# Autodesk Inventor assembly: main_assembly
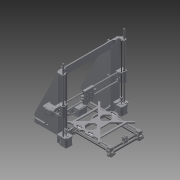
[picture p0: Inventor's stored thumbnail of the model, 180x180]
Saved by Autodesk Inventor 2015 SP2 (Build 190223200, 223)
## iProperties
Created: 2015-05-09
Part Number: main_assembly
Document SubType Name: Assembly
Designer: X
Author: X
## Documents named in this file (22)
- C:\Users\marc\Documents\GitHub\Prusa_i3\main_assembly.iam
- C:\Users\marc\Documents\GitHub\Prusa_i3\frame\platform_redrawn.ipt
- C:\Users\marc\Documents\GitHub\Prusa_i3\3d_printer_part\y-belt-holder.ipt
- C:\Users\marc\Documents\GitHub\Prusa_i3\chassis.iam
- C:\Users\marc\Documents\GitHub\Prusa_i3\Imported Components\NEMA 17 Stepper Motor Assembly\NEMA 17 Stepper Motor Assembly.iam
- C:\Users\marc\Documents\GitHub\Prusa_i3\standard_parts\LM8UU 8mm Linear Bearing.ipt
- C:\Users\marc\Documents\GitHub\Prusa_i3\main_frame_assem.iam
- C:\Users\marc\Documents\GitHub\Prusa_i3\standard_parts\ISO 7093 A\ISO 7093 A - ST 10 - 140 HV .ipt
- C:\Users\marc\Documents\GitHub\Prusa_i3\standard_parts\DIN 934\DIN 934 - M10 x 1.5.ipt
- C:\Users\marc\Documents\GitHub\Prusa_i3\standard_parts\DIN 84\DIN 84 - M3 x 16.ipt
- C:\Users\marc\Documents\GitHub\Prusa_i3\standard_parts\DIN 7985 (H)\DIN 7985 (H) - M3x18-H.ipt
- C:\Users\marc\Documents\GitHub\Prusa_i3\standard_parts\DIN 7985 (H)\DIN 7985 (H) - M3x16-H.ipt
- C:\Users\marc\Documents\GitHub\Prusa_i3\standard_parts\DIN 934\DIN 934 - M3.5 x 0.6.ipt
- C:\Users\marc\Documents\GitHub\Prusa_i3\Imported Components\coupler\coupler.ipt
- C:\Users\marc\Documents\GitHub\Prusa_i3\rod\smooth_rod_z_axis.ipt
- C:\Users\marc\Documents\GitHub\Prusa_i3\rod\threaded_rod_z_axis.ipt
- C:\Users\marc\Documents\GitHub\Prusa_i3\3d_printer_part\x-end-motor.ipt
- C:\Users\marc\Documents\GitHub\Prusa_i3\3d_printer_part\x-end-idler.ipt
- C:\Users\marc\Documents\GitHub\Prusa_i3\rod\smooth_rod_x_axis.ipt
- C:\Users\marc\Documents\GitHub\Prusa_i3\3d_printer_part\x-carriage.ipt
- C:\Users\marc\Documents\GitHub\Prusa_i3\frame\support1.ipt
- C:\Users\marc\Documents\GitHub\Prusa_i3\frame\support2.ipt
## Components (66 placed, 21 different names)
1. platform_redrawn:1 — Cylindrical:1, Cylindrical:2, Mate:1, Angle:1, Mate:3, Tangent:1, Tangent:2, Mate:4, Mate:5, Mate:27
2. y-belt-holder:1 — Cylindrical:1, Cylindrical:2, Mate:1
3. chassis:1 [sub-assembly] — Cylindrical:3, Cylindrical:4, Mate:2, Cylindrical:5, Cylindrical:6, Cylindrical:7, Angle:1, Mate:6, Mate:7, Cylindrical:8, Cylindrical:9, Cylindrical:10, Cylindrical:11, Cylindrical:12, Cylindrical:13, Cylindrical:14, Cylindrical:15, Cylindrical:16, Cylindrical:17, Mate:27, Flush:1, Mate:30
4. NEMA 17 Stepper Motor Assembly:1 [sub-assembly] — Cylindrical:3, Cylindrical:4, Mate:2
5. LM8UU 8mm Linear Bearing:1 — Cylindrical:6, Mate:3, Tangent:1, Tangent:2
6. LM8UU 8mm Linear Bearing:2 — Cylindrical:5, Mate:4
7. LM8UU 8mm Linear Bearing:3 — Cylindrical:7, Mate:5
8. main_frame_assem:1 [sub-assembly] — Cylindrical:8, Cylindrical:9, Mate:8, Mate:9, Mate:10, Mate:11, Mate:16, Cylindrical:18, Mate:17, Cylindrical:19, Mate:18, Cylindrical:20, Insert:1, Insert:2, Insert:3, Mate:19, Cylindrical:21, Mate:20, Cylindrical:22, Cylindrical:23, Mate:21, Mate:22, Mate:23, Mate:24, Mate:25, Mate:26, Insert:4, Insert:5, Insert:6, Insert:7, Insert:8, Insert:9, Insert:10, Insert:11, Insert:12, Insert:13, Insert:14, Insert:15, Insert:16, Insert:17, Insert:18, Insert:19, Insert:20, Cylindrical:26, Cylindrical:27, Mate:30, Mate:38, Mate:39, Mate:40, Mate:41, Mate:42, Mate:43
9. ISO 7093 A ST 10 - 140 HV - A:1 — Cylindrical:12, Mate:9, Mate:12
10. ISO 7093 A ST 10 - 140 HV - A:2 — Cylindrical:13, Mate:10, Mate:13
11. ISO 7093 A ST 10 - 140 HV - A:3 — Cylindrical:10, Mate:8, Mate:15
12. ISO 7093 A ST 10 - 140 HV - A:4 — Cylindrical:11, Mate:11, Mate:14
13. DIN 934 - replaced by DIN EN 24032/28673/28674 M10:1 — Cylindrical:14, Mate:12
14. DIN 934 - replaced by DIN EN 24032/28673/28674 M10:2 — Cylindrical:15, Mate:13
15. DIN 934 - replaced by DIN EN 24032/28673/28674 M10:3 — Cylindrical:17, Mate:15
16. DIN 934 - replaced by DIN EN 24032/28673/28674 M10:4 — Cylindrical:16, Mate:14
17. DIN 84 - replaced by DIN EN ISO 1207 M3 x 16:1 — Mate:16, Cylindrical:18
18. DIN 84 - replaced by DIN EN ISO 1207 M3 x 16:2 — Mate:17, Cylindrical:19
19. DIN 84 - replaced by DIN EN ISO 1207 M3 x 16:3 — Mate:18, Cylindrical:20
20. DIN 84 - replaced by DIN EN ISO 1207 M3 x 16:4 — Insert:1
21. DIN 84 - replaced by DIN EN ISO 1207 M3 x 16:5 — Insert:2
22. DIN 84 - replaced by DIN EN ISO 1207 M3 x 16:6 — Insert:3
23. NEMA 17 Stepper Motor Assembly:2 [sub-assembly] — Mate:19, Cylindrical:21, Cylindrical:24, Cylindrical:25, Mate:28, Mate:31, Mate:34
24. NEMA 17 Stepper Motor Assembly:3 [sub-assembly] — Mate:20, Cylindrical:22, Cylindrical:23, Mate:29, Cylindrical:28, Mate:32, Mate:33
25. DIN 7985 (H) M3x18-H:1 — Mate:21, Mate:22
26. DIN 7985 (H) M3x18-H:2 — Mate:23, Mate:24
27. DIN 7985 (H) M3x18-H:3 — Mate:25, Mate:26, Cylindrical:25
28. DIN 7985 (H) M3x18-H:4 — Insert:4
29. DIN 7985 (H) M3x18-H:5 — Insert:5
30. DIN 7985 (H) M3x18-H:6 — Insert:6
31. DIN 7985 (H) M3x16-H:1 — Insert:7
32. DIN 7985 (H) M3x16-H:2 — Insert:8
33. DIN 7985 (H) M3x16-H:3 — Insert:9
34. DIN 7985 (H) M3x16-H:4 — Insert:10
35. DIN 934 - replaced by DIN EN 24032/28673/28674 M3.5:1 — Insert:11
36. DIN 934 - replaced by DIN EN 24032/28673/28674 M3.5:2 — Insert:12
37. DIN 934 - replaced by DIN EN 24032/28673/28674 M3.5:3 — Insert:13
38. DIN 934 - replaced by DIN EN 24032/28673/28674 M3.5:4 — Insert:14
39. DIN 934 - replaced by DIN EN 24032/28673/28674 M3.5:5 — Insert:15
40. DIN 934 - replaced by DIN EN 24032/28673/28674 M3.5:6 — Insert:16
41. DIN 934 - replaced by DIN EN 24032/28673/28674 M3.5:7 — Insert:17
42. DIN 934 - replaced by DIN EN 24032/28673/28674 M3.5:8 — Insert:18
43. DIN 934 - replaced by DIN EN 24032/28673/28674 M3.5:9 — Insert:19
44. DIN 934 - replaced by DIN EN 24032/28673/28674 M3.5:10 — Insert:20
45. coupler:1 — Cylindrical:24, Mate:31, Cylindrical:30
46. smooth_rod_z_axis:1 — Cylindrical:26, Mate:28, Cylindrical:39
47. smooth_rod_z_axis:2 — Cylindrical:27, Mate:29, Cylindrical:35
48. coupler:2 — Cylindrical:28, Mate:32, Cylindrical:29
49. threaded_rod_z_axis:1 — Mate:33, Cylindrical:29, Cylindrical:37
50. threaded_rod_z_axis:2 — Mate:34, Cylindrical:30, Cylindrical:40
51. x-end-idler:1 — Cylindrical:33, Cylindrical:34, Flush:4, Flush:5, Cylindrical:35, Cylindrical:37, Cylindrical:41, Cylindrical:42, Mate:35, Mate:36
52. LM8UU 8mm Linear Bearing:4 — Cylindrical:32, Cylindrical:38, Flush:6, Cylindrical:39
53. LM8UU 8mm Linear Bearing:5 — Cylindrical:32, Flush:7
54. LM8UU 8mm Linear Bearing:6 — Cylindrical:34, Flush:4
55. LM8UU 8mm Linear Bearing:7 — Cylindrical:33, Flush:5
56. x-end-motor:1 — Cylindrical:38, Flush:6, Flush:7, Cylindrical:40, Cylindrical:43, Cylindrical:44, Mate:37, Cylindrical:45, Cylindrical:46
57. smooth_rod_x_axis:1 — Cylindrical:41, Cylindrical:44, Mate:35, Cylindrical:51
58. smooth_rod_x_axis:2 — Cylindrical:42, Cylindrical:43, Mate:36, Cylindrical:52
59. NEMA 17 Stepper Motor Assembly:4 [sub-assembly] — Mate:37, Cylindrical:45, Cylindrical:46
60. x-carriage:1 — Cylindrical:47, Cylindrical:48, Cylindrical:49, Cylindrical:50, Flush:8, Flush:9, Flush:10, Flush:11, Cylindrical:51, Cylindrical:52
61. LM8UU 8mm Linear Bearing:8 — Cylindrical:47, Flush:9
62. LM8UU 8mm Linear Bearing:9 — Cylindrical:48, Flush:8
63. LM8UU 8mm Linear Bearing:10 — Cylindrical:49, Flush:10
64. LM8UU 8mm Linear Bearing:11 — Cylindrical:50, Flush:11
65. support1:1 — Mate:38, Mate:39, Mate:40
66. support2:1 — Mate:41, Mate:42, Mate:43
## Relationships (125: CylindricalJoint 50, Mate 43, Insert 20, Flush 9, Tangent 2, Angle 1)
- Cylindrical:1: platform_redrawn:1 ↔ y-belt-holder:1
- Cylindrical:2: platform_redrawn:1 ↔ y-belt-holder:1
- Mate:1: platform_redrawn:1 ↔ y-belt-holder:1
- Cylindrical:3: chassis:1 ↔ NEMA 17 Stepper Motor Assembly:1
- Cylindrical:4: chassis:1 ↔ NEMA 17 Stepper Motor Assembly:1
- Mate:2: chassis:1 ↔ NEMA 17 Stepper Motor Assembly:1
- Cylindrical:5: chassis:1 ↔ LM8UU 8mm Linear Bearing:2
- Cylindrical:6: chassis:1 ↔ LM8UU 8mm Linear Bearing:1
- Cylindrical:7: chassis:1 ↔ LM8UU 8mm Linear Bearing:3
- Angle:1 (0 deg): platform_redrawn:1 ↔ chassis:1
- Mate:3 (3.5 mm): platform_redrawn:1 ↔ LM8UU 8mm Linear Bearing:1
- Tangent:1: platform_redrawn:1 ↔ LM8UU 8mm Linear Bearing:1
- Tangent:2: platform_redrawn:1 ↔ LM8UU 8mm Linear Bearing:1
- Mate:4 (3.5 mm): platform_redrawn:1 ↔ LM8UU 8mm Linear Bearing:2
- Mate:5 (3.5 mm): platform_redrawn:1 ↔ LM8UU 8mm Linear Bearing:3
- Mate:6: chassis:1
- Mate:7: chassis:1
- Cylindrical:8: chassis:1 ↔ main_frame_assem:1
- Cylindrical:9: chassis:1 ↔ main_frame_assem:1
- Cylindrical:10: chassis:1 ↔ ISO 7093 A ST 10 - 140 HV - A:3
- Cylindrical:11: chassis:1 ↔ ISO 7093 A ST 10 - 140 HV - A:4
- Cylindrical:12: chassis:1 ↔ ISO 7093 A ST 10 - 140 HV - A:1
- Cylindrical:13: chassis:1 ↔ ISO 7093 A ST 10 - 140 HV - A:2
- Mate:8: main_frame_assem:1 ↔ ISO 7093 A ST 10 - 140 HV - A:3
- Mate:9: main_frame_assem:1 ↔ ISO 7093 A ST 10 - 140 HV - A:1
- Mate:10: main_frame_assem:1 ↔ ISO 7093 A ST 10 - 140 HV - A:2
- Mate:11: main_frame_assem:1 ↔ ISO 7093 A ST 10 - 140 HV - A:4
- Cylindrical:14: chassis:1 ↔ DIN 934 - replaced by DIN EN 24032/28673/28674 M10:1
- Cylindrical:15: chassis:1 ↔ DIN 934 - replaced by DIN EN 24032/28673/28674 M10:2
- Cylindrical:16: chassis:1 ↔ DIN 934 - replaced by DIN EN 24032/28673/28674 M10:4
- Cylindrical:17: chassis:1 ↔ DIN 934 - replaced by DIN EN 24032/28673/28674 M10:3
- Mate:12: ISO 7093 A ST 10 - 140 HV - A:1 ↔ DIN 934 - replaced by DIN EN 24032/28673/28674 M10:1
- Mate:13: ISO 7093 A ST 10 - 140 HV - A:2 ↔ DIN 934 - replaced by DIN EN 24032/28673/28674 M10:2
- Mate:14: ISO 7093 A ST 10 - 140 HV - A:4 ↔ DIN 934 - replaced by DIN EN 24032/28673/28674 M10:4
- Mate:15: ISO 7093 A ST 10 - 140 HV - A:3 ↔ DIN 934 - replaced by DIN EN 24032/28673/28674 M10:3
- Mate:16: main_frame_assem:1 ↔ DIN 84 - replaced by DIN EN ISO 1207 M3 x 16:1
- Cylindrical:18: main_frame_assem:1 ↔ DIN 84 - replaced by DIN EN ISO 1207 M3 x 16:1
- Mate:17: main_frame_assem:1 ↔ DIN 84 - replaced by DIN EN ISO 1207 M3 x 16:2
- Cylindrical:19: main_frame_assem:1 ↔ DIN 84 - replaced by DIN EN ISO 1207 M3 x 16:2
- Mate:18: main_frame_assem:1 ↔ DIN 84 - replaced by DIN EN ISO 1207 M3 x 16:3
- Cylindrical:20: main_frame_assem:1 ↔ DIN 84 - replaced by DIN EN ISO 1207 M3 x 16:3
- Insert:1: main_frame_assem:1 ↔ DIN 84 - replaced by DIN EN ISO 1207 M3 x 16:4
- Insert:2: main_frame_assem:1 ↔ DIN 84 - replaced by DIN EN ISO 1207 M3 x 16:5
- Insert:3: main_frame_assem:1 ↔ DIN 84 - replaced by DIN EN ISO 1207 M3 x 16:6
- Mate:19: main_frame_assem:1 ↔ NEMA 17 Stepper Motor Assembly:2
- Cylindrical:21: main_frame_assem:1 ↔ NEMA 17 Stepper Motor Assembly:2
- Mate:20: main_frame_assem:1 ↔ NEMA 17 Stepper Motor Assembly:3
- Cylindrical:22: main_frame_assem:1 ↔ NEMA 17 Stepper Motor Assembly:3
- Cylindrical:23: main_frame_assem:1 ↔ NEMA 17 Stepper Motor Assembly:3
- Mate:21: main_frame_assem:1 ↔ DIN 7985 (H) M3x18-H:1
- Mate:22: main_frame_assem:1 ↔ DIN 7985 (H) M3x18-H:1
- Mate:23: main_frame_assem:1 ↔ DIN 7985 (H) M3x18-H:2
- Mate:24: main_frame_assem:1 ↔ DIN 7985 (H) M3x18-H:2
- Mate:25: main_frame_assem:1 ↔ DIN 7985 (H) M3x18-H:3
- Mate:26: main_frame_assem:1 ↔ DIN 7985 (H) M3x18-H:3
- Insert:4: main_frame_assem:1 ↔ DIN 7985 (H) M3x18-H:4
- Insert:5: main_frame_assem:1 ↔ DIN 7985 (H) M3x18-H:5
- Insert:6: main_frame_assem:1 ↔ DIN 7985 (H) M3x18-H:6
- Insert:7: main_frame_assem:1 ↔ DIN 7985 (H) M3x16-H:1
- Insert:8: main_frame_assem:1 ↔ DIN 7985 (H) M3x16-H:2
- Insert:9: main_frame_assem:1 ↔ DIN 7985 (H) M3x16-H:3
- Insert:10: main_frame_assem:1 ↔ DIN 7985 (H) M3x16-H:4
- Insert:11: main_frame_assem:1 ↔ DIN 934 - replaced by DIN EN 24032/28673/28674 M3.5:1
- Insert:12: main_frame_assem:1 ↔ DIN 934 - replaced by DIN EN 24032/28673/28674 M3.5:2
- Insert:13: main_frame_assem:1 ↔ DIN 934 - replaced by DIN EN 24032/28673/28674 M3.5:3
- Insert:14: main_frame_assem:1 ↔ DIN 934 - replaced by DIN EN 24032/28673/28674 M3.5:4
- Insert:15: main_frame_assem:1 ↔ DIN 934 - replaced by DIN EN 24032/28673/28674 M3.5:5
- Insert:16: main_frame_assem:1 ↔ DIN 934 - replaced by DIN EN 24032/28673/28674 M3.5:6
- Insert:17: main_frame_assem:1 ↔ DIN 934 - replaced by DIN EN 24032/28673/28674 M3.5:7
- Insert:18: main_frame_assem:1 ↔ DIN 934 - replaced by DIN EN 24032/28673/28674 M3.5:8
- Insert:19: main_frame_assem:1 ↔ DIN 934 - replaced by DIN EN 24032/28673/28674 M3.5:9
- Insert:20: main_frame_assem:1 ↔ DIN 934 - replaced by DIN EN 24032/28673/28674 M3.5:10
- Cylindrical:24: NEMA 17 Stepper Motor Assembly:2 ↔ coupler:1
- Cylindrical:25: NEMA 17 Stepper Motor Assembly:2 ↔ DIN 7985 (H) M3x18-H:3
- Mate:27 (60 mm): platform_redrawn:1 ↔ chassis:1
- Flush:1: chassis:1
- Cylindrical:26: main_frame_assem:1 ↔ smooth_rod_z_axis:1
- Mate:28: NEMA 17 Stepper Motor Assembly:2 ↔ smooth_rod_z_axis:1
- Cylindrical:27: main_frame_assem:1 ↔ smooth_rod_z_axis:2
- Mate:29: NEMA 17 Stepper Motor Assembly:3 ↔ smooth_rod_z_axis:2
- Mate:30 (100 mm): chassis:1 ↔ main_frame_assem:1
- Mate:31 (12 mm): NEMA 17 Stepper Motor Assembly:2 ↔ coupler:1
- Cylindrical:28: NEMA 17 Stepper Motor Assembly:3 ↔ coupler:2
- Mate:32 (12 mm): NEMA 17 Stepper Motor Assembly:3 ↔ coupler:2
- Mate:33: NEMA 17 Stepper Motor Assembly:3 ↔ threaded_rod_z_axis:1
- Cylindrical:29: coupler:2 ↔ threaded_rod_z_axis:1
- Mate:34: NEMA 17 Stepper Motor Assembly:2 ↔ threaded_rod_z_axis:2
- Cylindrical:30: coupler:1 ↔ threaded_rod_z_axis:2
- Cylindrical:32: LM8UU 8mm Linear Bearing:4 ↔ LM8UU 8mm Linear Bearing:5
- Cylindrical:33: x-end-idler:1 ↔ LM8UU 8mm Linear Bearing:7
- Cylindrical:34: x-end-idler:1 ↔ LM8UU 8mm Linear Bearing:6
- Flush:4: x-end-idler:1 ↔ LM8UU 8mm Linear Bearing:6
- Flush:5: x-end-idler:1 ↔ LM8UU 8mm Linear Bearing:7
- Cylindrical:35: smooth_rod_z_axis:2 ↔ x-end-idler:1
- Cylindrical:37: threaded_rod_z_axis:1 ↔ x-end-idler:1
- Cylindrical:38: LM8UU 8mm Linear Bearing:4 ↔ x-end-motor:1
- Flush:6: LM8UU 8mm Linear Bearing:4 ↔ x-end-motor:1
- Flush:7: LM8UU 8mm Linear Bearing:5 ↔ x-end-motor:1
- Cylindrical:39: smooth_rod_z_axis:1 ↔ LM8UU 8mm Linear Bearing:4
- Cylindrical:40: threaded_rod_z_axis:2 ↔ x-end-motor:1
- Cylindrical:41: x-end-idler:1 ↔ smooth_rod_x_axis:1
- Cylindrical:42: x-end-idler:1 ↔ smooth_rod_x_axis:2
- Cylindrical:43: x-end-motor:1 ↔ smooth_rod_x_axis:2
- Cylindrical:44: x-end-motor:1 ↔ smooth_rod_x_axis:1
- Mate:35 (18.5 mm): x-end-idler:1 ↔ smooth_rod_x_axis:1
- Mate:36 (18.5 mm): x-end-idler:1 ↔ smooth_rod_x_axis:2
- Mate:37: x-end-motor:1 ↔ NEMA 17 Stepper Motor Assembly:4
- Cylindrical:45: x-end-motor:1 ↔ NEMA 17 Stepper Motor Assembly:4
- Cylindrical:46: x-end-motor:1 ↔ NEMA 17 Stepper Motor Assembly:4
- Cylindrical:47: x-carriage:1 ↔ LM8UU 8mm Linear Bearing:8
- Cylindrical:48: x-carriage:1 ↔ LM8UU 8mm Linear Bearing:9
- Cylindrical:49: x-carriage:1 ↔ LM8UU 8mm Linear Bearing:10
- Cylindrical:50: x-carriage:1 ↔ LM8UU 8mm Linear Bearing:11
- Flush:8: x-carriage:1 ↔ LM8UU 8mm Linear Bearing:9
- Flush:9: x-carriage:1 ↔ LM8UU 8mm Linear Bearing:8
- Flush:10: x-carriage:1 ↔ LM8UU 8mm Linear Bearing:10
- Flush:11: x-carriage:1 ↔ LM8UU 8mm Linear Bearing:11
- Cylindrical:51: smooth_rod_x_axis:1 ↔ x-carriage:1
- Cylindrical:52: smooth_rod_x_axis:2 ↔ x-carriage:1
- Mate:38: main_frame_assem:1 ↔ support1:1
- Mate:39: main_frame_assem:1 ↔ support1:1
- Mate:40: main_frame_assem:1 ↔ support1:1
- Mate:41: main_frame_assem:1 ↔ support2:1
- Mate:42: main_frame_assem:1 ↔ support2:1
- Mate:43: main_frame_assem:1 ↔ support2:1
